# Autodesk Inventor assembly: final model 3.1
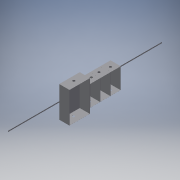
[picture p0: Inventor's stored thumbnail of the model, 180x180]
Saved by Autodesk Inventor 2019 (Build 230136000, 136)
## iProperties
Created: 2019-10-17
Part Number: final model 3.1
Document SubType Name: Assembly
Designer: DELL
Author: DELL
## Documents named in this file (5)
- D:\exploration\virtual model\final model 3.1.iam
- D:\exploration\virtual model\Assembly2.iam
- D:\exploration\virtual model\new box.iam
- D:\exploration\virtual model\new assembly 3.ipt
- D:\exploration\virtual model\rod2.0.ipt
## Components (13 placed, 4 different names)
1. Assembly2:1 [sub-assembly] — Rigid:1, Rigid:2, Rigid:7, Rigid:8
2. new box:1 [sub-assembly] — Rigid:7, Rigid:11
3. new assembly 3:1 — Rigid:2
4. new assembly 3:2 — Rigid:1
5. Assembly2:2 [sub-assembly] — Rigid:8, Rigid:9
6. new assembly 3:3
7. new assembly 3:4
8. Assembly2:3 [sub-assembly] — Rigid:9, Rigid:10, Rigid:12
9. new assembly 3:5
10. new assembly 3:6
11. rod2.0:1 — Rigid:10
12. rod2.0:2 — Rigid:11
13. rod2.0:3 — Rigid:12
## Relationships (12: WeldJoint 12)
- Rigid:1 [WeldJoint]: Assembly2:1 ↔ new assembly 3:2
- Rigid:2 [WeldJoint]: Assembly2:1 ↔ new assembly 3:1
- [WeldJoint]: Assembly2:2 ↔ new assembly 3:4
- [WeldJoint]: Assembly2:2 ↔ new assembly 3:3
- [WeldJoint]: Assembly2:3 ↔ new assembly 3:6
- [WeldJoint]: Assembly2:3 ↔ new assembly 3:5
- Rigid:7 [WeldJoint]: Assembly2:1 ↔ new box:1
- Rigid:8 [WeldJoint]: Assembly2:1 ↔ Assembly2:2
- Rigid:9 [WeldJoint]: Assembly2:2 ↔ Assembly2:3
- Rigid:10 [WeldJoint]: Assembly2:3 ↔ rod2.0:1
- Rigid:11 [WeldJoint]: new box:1 ↔ rod2.0:2
- Rigid:12 [WeldJoint]: Assembly2:3 ↔ rod2.0:3
## Named parameters: d2_d0 = 0 mm, d3_d1 = 0 mm, d4_d0 = 0 mm, d5_d1 = 0 mm
